# Autodesk Inventor assembly: Trolley
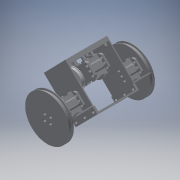
[picture p0: Inventor's stored thumbnail of the model, 180x180]
Saved by Autodesk Inventor 2016 (Build 200138000, 138)
## iProperties
Created: 2016-04-01
Part Number: Trolley
Document SubType Name: Assembly
Designer: mkepler
Author: mkepler
## Documents named in this file (10)
- C:\Users\mkepler\Google Drive\Michael Kepler\College\ECE\ECE 590\Project 2\Inventor Files\Trolley\Trolley.iam
- C:\Users\mkepler\Google Drive\Michael Kepler\College\ECE\ECE 590\Project 2\Inventor Files\Trolley\TrolleyBottomPlate.ipt
- C:\Users\mkepler\Google Drive\Michael Kepler\College\ECE\ECE 590\Project 2\Inventor Files\Trolley\TrolleyRightPlate.ipt
- C:\Users\mkepler\Google Drive\Michael Kepler\College\ECE\ECE 590\Project 2\Inventor Files\Trolley\TrolleyLeftPlate.ipt
- C:\Users\mkepler\Google Drive\Michael Kepler\College\ECE\ECE 590\Project 2\Inventor Files\PegLarge.ipt
- C:\Users\mkepler\Google Drive\Michael Kepler\College\ECE\ECE 590\Project 2\Inventor Files\xl320Servo.ipt
- C:\Users\mkepler\Google Drive\Michael Kepler\College\ECE\ECE 590\Project 2\Inventor Files\Trolley\TrolleyTopPlate.ipt
- C:\Users\mkepler\Google Drive\Michael Kepler\College\ECE\ECE 590\Project 2\Inventor Files\Trolley\XLRotorWheel.ipt
- C:\Users\mkepler\Google Drive\Michael Kepler\College\ECE\ECE 590\Project 2\Inventor Files\Trolley\SingleAxialWheel.ipt
- C:\Users\mkepler\Google Drive\Michael Kepler\College\ECE\ECE 590\Project 2\Inventor Files\Trolley\LargeWheel.ipt
## Components (15 placed, 9 different names)
1. TrolleyBottomPlate:1 — Insert:1, Insert:2, Insert:3, Insert:4
2. TrolleyRightPlate:1 — Insert:1, Insert:2, Insert:6, Insert:9, Insert:14, Mate:1, Insert:16
3. TrolleyLeftPlate:1 — Insert:3, Insert:4, Insert:7, Insert:8, Insert:10, Insert:11, Insert:15
4. PegLarge:1 — Insert:6
5. PegLarge:2 — Insert:7, Insert:13
6. PegLarge:3 — Insert:9
7. PegLarge:4 — Insert:8, Insert:12
8. xl320Servo:1 — Insert:10, Insert:11, Insert:20, Insert:21
9. xl320Servo:2 — Insert:12, Insert:13, Insert:17, Insert:18, Insert:19
10. xl320Servo:3 — Insert:14, Mate:1, Insert:22, Mate:2
11. TrolleyTopPlate:1 — Insert:15, Insert:16
12. XLRotorWheel:1 — Insert:17, Insert:19
13. SingleAxialWheel:1 — Insert:18
14. LargeWheel:1 — Insert:20, Insert:21
15. LargeWheel:2 — Insert:22, Mate:2
## Relationships (23: Insert 21, Mate 2)
- Insert:1: TrolleyBottomPlate:1 ↔ TrolleyRightPlate:1
- Insert:2: TrolleyBottomPlate:1 ↔ TrolleyRightPlate:1
- Insert:3: TrolleyBottomPlate:1 ↔ TrolleyLeftPlate:1
- Insert:4: TrolleyBottomPlate:1 ↔ TrolleyLeftPlate:1
- Insert:6: TrolleyRightPlate:1 ↔ PegLarge:1
- Insert:7: TrolleyLeftPlate:1 ↔ PegLarge:2
- Insert:8: TrolleyLeftPlate:1 ↔ PegLarge:4
- Insert:9: TrolleyRightPlate:1 ↔ PegLarge:3
- Insert:10: TrolleyLeftPlate:1 ↔ xl320Servo:1
- Insert:11: TrolleyLeftPlate:1 ↔ xl320Servo:1
- Insert:12: PegLarge:4 ↔ xl320Servo:2
- Insert:13: PegLarge:2 ↔ xl320Servo:2
- Insert:14: TrolleyRightPlate:1 ↔ xl320Servo:3
- Mate:1: TrolleyRightPlate:1 ↔ xl320Servo:3
- Insert:15: TrolleyLeftPlate:1 ↔ TrolleyTopPlate:1
- Insert:16: TrolleyRightPlate:1 ↔ TrolleyTopPlate:1
- Insert:17: xl320Servo:2 ↔ XLRotorWheel:1
- Insert:18: xl320Servo:2 ↔ SingleAxialWheel:1
- Insert:19: xl320Servo:2 ↔ XLRotorWheel:1
- Insert:20: xl320Servo:1 ↔ LargeWheel:1
- Insert:21: xl320Servo:1 ↔ LargeWheel:1
- Insert:22: xl320Servo:3 ↔ LargeWheel:2
- Mate:2: xl320Servo:3 ↔ LargeWheel:2
